# Autodesk Inventor assembly: completeCase
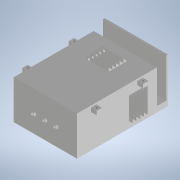
[picture p0: Inventor's stored thumbnail of the model, 180x180]
Saved by Autodesk Inventor 2022.6 (Build 266554010, 554A)
## iProperties
Created: 2025-03-20
Part Number: completeCase
Document SubType Name: Assembly
Designer: khinm
Author: khinm
## Documents named in this file (3)
- C:\Users\khinm\Downloads\CAD\toolkit_controllerCaseDesign\completeCase.iam
- C:\Users\khinm\Downloads\CAD\toolkit_controllerCaseDesign\caseBody_basePlate.iam
- C:\Users\khinm\Downloads\CAD\toolkit_controllerCaseDesign\caseDoor_rubberSeal.iam
## Components (2 placed, 2 different names)
1. caseBody_basePlate:1 [sub-assembly] — Flush:1, Flush:2, Flush:3, Mate:1
2. caseDoor_rubberSeal:1 [sub-assembly] — Flush:1, Flush:2, Flush:3, Mate:1
## Relationships (4: Flush 3, Mate 1)
- Flush:1: caseBody_basePlate:1 ↔ caseDoor_rubberSeal:1
- Flush:2: caseBody_basePlate:1 ↔ caseDoor_rubberSeal:1
- Flush:3: caseBody_basePlate:1 ↔ caseDoor_rubberSeal:1
- Mate:1: caseBody_basePlate:1 ↔ caseDoor_rubberSeal:1
